# Autodesk Inventor assembly: T4DB 170
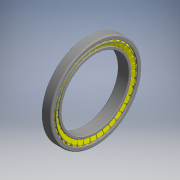
[picture p0: Inventor's stored thumbnail of the model, 180x180]
Saved by Autodesk Inventor 2017.3 (Build 213256000, 256)
## iProperties
Category: PARTsolutions
Company: SKF
Part Number: T4DB 170
Catalog Web Link: www.cadenas.de
Description: BT1_001_101-Tapered roller bearings, single row
Vendor: SKF
Document SubType Name: Assembly
Designer: partserver
Manufacturer: SKF
Mass: 3439 g
Surface Area: 1785.69 cm^2
Volume: 432.234 cm^3
Density: 7.95634 g/cm^3
Title: T4DB 170
Author: Cadenas PARTsolutions
Comments: Tapered roller bearings, single row
PSOL_IDENT_0: {$CADENAS_DATA\23d-libs\skf\bearings_units_and_housings\roller_bearings\tapered_roller_bearings\tape
PSOL_IDENT_1: red_roller_bearings_single_row\bt1_001_101.prj},177 {VTYP=3D},{STYP=ASSTAB},{NB=T4DB 170},{LINA=T4DB
PSOL_IDENT_2: 170},{NN=BT1_001_101},{DATE=23.12.2020 07:01:44},{GEOMDATE=30.11.2020 07:39:16},{VERSION=},{LINEID=
PSOL_IDENT_3: 4320},{WBVAR=},{WBNUMERIC=}  {NB=T4DB 170},{LINA=T4DB 170},{KT=DUMMY},{DESIGNATION=T4DB 170},{DD=170
PSOL_IDENT_4: .000},{D=230.000},{T=32.000},{DD1=197.5000},{D1=MIN},{ALPHA=17.100},{RANGLE=2.500},{IRA=14.600},{B=3
PSOL_IDENT_5: 0.000},{C=23.000},{C1=MIN},{R12=3.0},{R34=3.0},{AA=44.29541},{PITCH=200.033},{DW=16.450},{LW=21.500}
PSOL_IDENT_6: ,{DDAMAX=182},{DDAMIN=184.5},{DAMIN=215},{DAMAX=216.0},{DBMIN=223},{CA=6},{CB=9.0},{RA=3.0},{RB=3.0}
PSOL_IDENT_7: ,{LOAD1=307.000},{LOAD2=440.000},{LOAD3=43.000},{SPEED1=2000},{SPEED2=2600},{EE=0.46},{Y=1.30},{Y0=0
PSOL_IDENT_8: .7},{Y1=0},{X1=1},{X2=0.4},{X0=0.5},{Z=37},{II=1},{R1=0.00000231},{R2=10.9},{S1=0.019},{S2=2},{KZ=6}
PSOL_IDENT_9: ,{KL=0.7},{BF=2},{MASS=3.439},{DESIGN=trb1},{HELP=0.000},{PPATH=parts/bt1_001_101_asmtpl.prj},{SUPPR
PSOL_IDENT_10: ESS=N},{A4=200000},{A15=350000},{BEARING=T4DB 170},{A8=300000},{POPULAR=}
NB: T4DB 170
NN: BT1_001_101
NT: Tapered roller bearings, single row
NBSYN: $DESIGNATION.
LINA: T4DB 170
CATALOG: SKF
DESIGNATION: T4DB 170
DD: 170
D: 230
T: 32
LOAD1: 307
LOAD2: 440
LOAD3: 43
SPEED1: 2000
SPEED2: 2600
A4: 200000
A15: 350000
BEARING: T4DB 170
A8: 300000
SUPPLIER: SKF
ARTICLENO: T4DB 170
BOMINFO: T4DB 170
CREATOR: CADENAS GmbH
## Documents named in this file (5)
- e:\temp\worker_20\temp\exporttempdir_7356_2_3SxGk\format_0\T4DB 170.iam
- e:\temp\worker_20\temp\exporttempdir_7356_2_3SxGk\format_0\T4DB 170_ir.ipt
- e:\temp\worker_20\temp\exporttempdir_7356_2_3SxGk\format_0\T4DB 170_cage.ipt
- e:\temp\worker_20\temp\exporttempdir_7356_2_3SxGk\format_0\T4DB 170_r.ipt
- e:\temp\worker_20\temp\exporttempdir_7356_2_3SxGk\format_0\T4DB 170_or.ipt
## Components (40 placed, 4 different names)
1. T4DB 170_ir:1
2. T4DB 170_cage:1 — roller1_XY@2 <-> roller_XY@3, roller1_Z@2 <-> roller_Z@3, roller1_YZ@2 <-> roller_YZ@3, roller2_XY@2 <-> roller_XY@4, roller2_Z@2 <-> roller_Z@4, roller2_YZ@2 <-> roller_YZ@4, roller3_XY@2 <-> roller_XY@5, roller3_Z@2 <-> roller_Z@5, roller3_YZ@2 <-> roller_YZ@5, roller4_XY@2 <-> roller_XY@6, roller4_Z@2 <-> roller_Z@6, roller4_YZ@2 <-> roller_YZ@6, roller5_XY@2 <-> roller_XY@7, roller5_Z@2 <-> roller_Z@7, roller5_YZ@2 <-> roller_YZ@7, roller6_XY@2 <-> roller_XY@8, roller6_Z@2 <-> roller_Z@8, roller6_YZ@2 <-> roller_YZ@8, roller7_XY@2 <-> roller_XY@9, roller7_Z@2 <-> roller_Z@9, roller7_YZ@2 <-> roller_YZ@9, roller8_XY@2 <-> roller_XY@10, roller8_Z@2 <-> roller_Z@10, roller8_YZ@2 <-> roller_YZ@10, roller9_XY@2 <-> roller_XY@11, roller9_Z@2 <-> roller_Z@11, roller9_YZ@2 <-> roller_YZ@11, roller10_XY@2 <-> roller_XY@12, roller10_Z@2 <-> roller_Z@12, roller10_YZ@2 <-> roller_YZ@12, roller11_XY@2 <-> roller_XY@13, roller11_Z@2 <-> roller_Z@13, roller11_YZ@2 <-> roller_YZ@13, roller12_XY@2 <-> roller_XY@14, roller12_Z@2 <-> roller_Z@14, roller12_YZ@2 <-> roller_YZ@14, roller13_XY@2 <-> roller_XY@15, roller13_Z@2 <-> roller_Z@15, roller13_YZ@2 <-> roller_YZ@15, roller14_XY@2 <-> roller_XY@16, roller14_Z@2 <-> roller_Z@16, roller14_YZ@2 <-> roller_YZ@16, roller15_XY@2 <-> roller_XY@17, roller15_Z@2 <-> roller_Z@17, roller15_YZ@2 <-> roller_YZ@17, roller16_XY@2 <-> roller_XY@18, roller16_Z@2 <-> roller_Z@18, roller16_YZ@2 <-> roller_YZ@18, roller17_XY@2 <-> roller_XY@19, roller17_Z@2 <-> roller_Z@19, roller17_YZ@2 <-> roller_YZ@19, roller18_XY@2 <-> roller_XY@20, roller18_Z@2 <-> roller_Z@20, roller18_YZ@2 <-> roller_YZ@20, roller19_XY@2 <-> roller_XY@21, roller19_Z@2 <-> roller_Z@21, roller19_YZ@2 <-> roller_YZ@21, roller20_XY@2 <-> roller_XY@22, roller20_Z@2 <-> roller_Z@22, roller20_YZ@2 <-> roller_YZ@22, roller21_XY@2 <-> roller_XY@23, roller21_Z@2 <-> roller_Z@23, roller21_YZ@2 <-> roller_YZ@23, roller22_XY@2 <-> roller_XY@24, roller22_Z@2 <-> roller_Z@24, roller22_YZ@2 <-> roller_YZ@24, roller23_XY@2 <-> roller_XY@25, roller23_Z@2 <-> roller_Z@25, roller23_YZ@2 <-> roller_YZ@25, roller24_XY@2 <-> roller_XY@26, roller24_Z@2 <-> roller_Z@26, roller24_YZ@2 <-> roller_YZ@26, roller25_XY@2 <-> roller_XY@27, roller25_Z@2 <-> roller_Z@27, roller25_YZ@2 <-> roller_YZ@27, roller26_XY@2 <-> roller_XY@28, roller26_Z@2 <-> roller_Z@28, roller26_YZ@2 <-> roller_YZ@28, roller27_XY@2 <-> roller_XY@29, roller27_Z@2 <-> roller_Z@29, roller27_YZ@2 <-> roller_YZ@29, roller28_XY@2 <-> roller_XY@30, roller28_Z@2 <-> roller_Z@30, roller28_YZ@2 <-> roller_YZ@30, roller29_XY@2 <-> roller_XY@31, roller29_Z@2 <-> roller_Z@31, roller29_YZ@2 <-> roller_YZ@31, roller30_XY@2 <-> roller_XY@32, roller30_Z@2 <-> roller_Z@32, roller30_YZ@2 <-> roller_YZ@32, roller31_XY@2 <-> roller_XY@33, roller31_Z@2 <-> roller_Z@33, roller31_YZ@2 <-> roller_YZ@33, roller32_XY@2 <-> roller_XY@34, roller32_Z@2 <-> roller_Z@34, roller32_YZ@2 <-> roller_YZ@34, roller33_XY@2 <-> roller_XY@35, roller33_Z@2 <-> roller_Z@35, roller33_YZ@2 <-> roller_YZ@35, roller34_XY@2 <-> roller_XY@36, roller34_Z@2 <-> roller_Z@36, roller34_YZ@2 <-> roller_YZ@36, roller35_XY@2 <-> roller_XY@37, roller35_Z@2 <-> roller_Z@37, roller35_YZ@2 <-> roller_YZ@37, roller36_XY@2 <-> roller_XY@38, roller36_Z@2 <-> roller_Z@38, roller36_YZ@2 <-> roller_YZ@38, roller37_XY@2 <-> roller_XY@39, roller37_Z@2 <-> roller_Z@39, roller37_YZ@2 <-> roller_YZ@39
3. T4DB 170_r:1 — roller1_XY@2 <-> roller_XY@3, roller1_Z@2 <-> roller_Z@3, roller1_YZ@2 <-> roller_YZ@3
4. T4DB 170_r:2 — roller2_XY@2 <-> roller_XY@4, roller2_Z@2 <-> roller_Z@4, roller2_YZ@2 <-> roller_YZ@4
5. T4DB 170_r:3 — roller3_XY@2 <-> roller_XY@5, roller3_Z@2 <-> roller_Z@5, roller3_YZ@2 <-> roller_YZ@5
6. T4DB 170_r:4 — roller4_XY@2 <-> roller_XY@6, roller4_Z@2 <-> roller_Z@6, roller4_YZ@2 <-> roller_YZ@6
7. T4DB 170_r:5 — roller5_XY@2 <-> roller_XY@7, roller5_Z@2 <-> roller_Z@7, roller5_YZ@2 <-> roller_YZ@7
8. T4DB 170_r:6 — roller6_XY@2 <-> roller_XY@8, roller6_Z@2 <-> roller_Z@8, roller6_YZ@2 <-> roller_YZ@8
9. T4DB 170_r:7 — roller7_XY@2 <-> roller_XY@9, roller7_Z@2 <-> roller_Z@9, roller7_YZ@2 <-> roller_YZ@9
10. T4DB 170_r:8 — roller8_XY@2 <-> roller_XY@10, roller8_Z@2 <-> roller_Z@10, roller8_YZ@2 <-> roller_YZ@10
11. T4DB 170_r:9 — roller9_XY@2 <-> roller_XY@11, roller9_Z@2 <-> roller_Z@11, roller9_YZ@2 <-> roller_YZ@11
12. T4DB 170_r:10 — roller10_XY@2 <-> roller_XY@12, roller10_Z@2 <-> roller_Z@12, roller10_YZ@2 <-> roller_YZ@12
13. T4DB 170_r:11 — roller11_XY@2 <-> roller_XY@13, roller11_Z@2 <-> roller_Z@13, roller11_YZ@2 <-> roller_YZ@13
14. T4DB 170_r:12 — roller12_XY@2 <-> roller_XY@14, roller12_Z@2 <-> roller_Z@14, roller12_YZ@2 <-> roller_YZ@14
15. T4DB 170_r:13 — roller13_XY@2 <-> roller_XY@15, roller13_Z@2 <-> roller_Z@15, roller13_YZ@2 <-> roller_YZ@15
16. T4DB 170_r:14 — roller14_XY@2 <-> roller_XY@16, roller14_Z@2 <-> roller_Z@16, roller14_YZ@2 <-> roller_YZ@16
17. T4DB 170_r:15 — roller15_XY@2 <-> roller_XY@17, roller15_Z@2 <-> roller_Z@17, roller15_YZ@2 <-> roller_YZ@17
18. T4DB 170_r:16 — roller16_XY@2 <-> roller_XY@18, roller16_Z@2 <-> roller_Z@18, roller16_YZ@2 <-> roller_YZ@18
19. T4DB 170_r:17 — roller17_XY@2 <-> roller_XY@19, roller17_Z@2 <-> roller_Z@19, roller17_YZ@2 <-> roller_YZ@19
20. T4DB 170_r:18 — roller18_XY@2 <-> roller_XY@20, roller18_Z@2 <-> roller_Z@20, roller18_YZ@2 <-> roller_YZ@20
21. T4DB 170_r:19 — roller19_XY@2 <-> roller_XY@21, roller19_Z@2 <-> roller_Z@21, roller19_YZ@2 <-> roller_YZ@21
22. T4DB 170_r:20 — roller20_XY@2 <-> roller_XY@22, roller20_Z@2 <-> roller_Z@22, roller20_YZ@2 <-> roller_YZ@22
23. T4DB 170_r:21 — roller21_XY@2 <-> roller_XY@23, roller21_Z@2 <-> roller_Z@23, roller21_YZ@2 <-> roller_YZ@23
24. T4DB 170_r:22 — roller22_XY@2 <-> roller_XY@24, roller22_Z@2 <-> roller_Z@24, roller22_YZ@2 <-> roller_YZ@24
25. T4DB 170_r:23 — roller23_XY@2 <-> roller_XY@25, roller23_Z@2 <-> roller_Z@25, roller23_YZ@2 <-> roller_YZ@25
26. T4DB 170_r:24 — roller24_XY@2 <-> roller_XY@26, roller24_Z@2 <-> roller_Z@26, roller24_YZ@2 <-> roller_YZ@26
27. T4DB 170_r:25 — roller25_XY@2 <-> roller_XY@27, roller25_Z@2 <-> roller_Z@27, roller25_YZ@2 <-> roller_YZ@27
28. T4DB 170_r:26 — roller26_XY@2 <-> roller_XY@28, roller26_Z@2 <-> roller_Z@28, roller26_YZ@2 <-> roller_YZ@28
29. T4DB 170_r:27 — roller27_XY@2 <-> roller_XY@29, roller27_Z@2 <-> roller_Z@29, roller27_YZ@2 <-> roller_YZ@29
30. T4DB 170_r:28 — roller28_XY@2 <-> roller_XY@30, roller28_Z@2 <-> roller_Z@30, roller28_YZ@2 <-> roller_YZ@30
31. T4DB 170_r:29 — roller29_XY@2 <-> roller_XY@31, roller29_Z@2 <-> roller_Z@31, roller29_YZ@2 <-> roller_YZ@31
32. T4DB 170_r:30 — roller30_XY@2 <-> roller_XY@32, roller30_Z@2 <-> roller_Z@32, roller30_YZ@2 <-> roller_YZ@32
33. T4DB 170_r:31 — roller31_XY@2 <-> roller_XY@33, roller31_Z@2 <-> roller_Z@33, roller31_YZ@2 <-> roller_YZ@33
34. T4DB 170_r:32 — roller32_XY@2 <-> roller_XY@34, roller32_Z@2 <-> roller_Z@34, roller32_YZ@2 <-> roller_YZ@34
35. T4DB 170_r:33 — roller33_XY@2 <-> roller_XY@35, roller33_Z@2 <-> roller_Z@35, roller33_YZ@2 <-> roller_YZ@35
36. T4DB 170_r:34 — roller34_XY@2 <-> roller_XY@36, roller34_Z@2 <-> roller_Z@36, roller34_YZ@2 <-> roller_YZ@36
37. T4DB 170_r:35 — roller35_XY@2 <-> roller_XY@37, roller35_Z@2 <-> roller_Z@37, roller35_YZ@2 <-> roller_YZ@37
38. T4DB 170_r:36 — roller36_XY@2 <-> roller_XY@38, roller36_Z@2 <-> roller_Z@38, roller36_YZ@2 <-> roller_YZ@38
39. T4DB 170_r:37 — roller37_XY@2 <-> roller_XY@39, roller37_Z@2 <-> roller_Z@39, roller37_YZ@2 <-> roller_YZ@39
40. T4DB 170_or:1
## Relationships (111: Mate 74, Angle 37)
- roller1_XY@2 <-> roller_XY@3 [Mate]: T4DB 170_cage:1 ↔ T4DB 170_r:1
- roller1_Z@2 <-> roller_Z@3 [Mate]: T4DB 170_cage:1 ↔ T4DB 170_r:1
- roller1_YZ@2 <-> roller_YZ@3 [Angle] (0 deg): T4DB 170_cage:1 ↔ T4DB 170_r:1
- roller2_XY@2 <-> roller_XY@4 [Mate]: T4DB 170_cage:1 ↔ T4DB 170_r:2
- roller2_Z@2 <-> roller_Z@4 [Mate]: T4DB 170_cage:1 ↔ T4DB 170_r:2
- roller2_YZ@2 <-> roller_YZ@4 [Angle] (0 deg): T4DB 170_cage:1 ↔ T4DB 170_r:2
- roller3_XY@2 <-> roller_XY@5 [Mate]: T4DB 170_cage:1 ↔ T4DB 170_r:3
- roller3_Z@2 <-> roller_Z@5 [Mate]: T4DB 170_cage:1 ↔ T4DB 170_r:3
- roller3_YZ@2 <-> roller_YZ@5 [Angle] (0 deg): T4DB 170_cage:1 ↔ T4DB 170_r:3
- roller4_XY@2 <-> roller_XY@6 [Mate]: T4DB 170_cage:1 ↔ T4DB 170_r:4
- roller4_Z@2 <-> roller_Z@6 [Mate]: T4DB 170_cage:1 ↔ T4DB 170_r:4
- roller4_YZ@2 <-> roller_YZ@6 [Angle] (0 deg): T4DB 170_cage:1 ↔ T4DB 170_r:4
- roller5_XY@2 <-> roller_XY@7 [Mate]: T4DB 170_cage:1 ↔ T4DB 170_r:5
- roller5_Z@2 <-> roller_Z@7 [Mate]: T4DB 170_cage:1 ↔ T4DB 170_r:5
- roller5_YZ@2 <-> roller_YZ@7 [Angle] (0 deg): T4DB 170_cage:1 ↔ T4DB 170_r:5
- roller6_XY@2 <-> roller_XY@8 [Mate]: T4DB 170_cage:1 ↔ T4DB 170_r:6
- roller6_Z@2 <-> roller_Z@8 [Mate]: T4DB 170_cage:1 ↔ T4DB 170_r:6
- roller6_YZ@2 <-> roller_YZ@8 [Angle] (0 deg): T4DB 170_cage:1 ↔ T4DB 170_r:6
- roller7_XY@2 <-> roller_XY@9 [Mate]: T4DB 170_cage:1 ↔ T4DB 170_r:7
- roller7_Z@2 <-> roller_Z@9 [Mate]: T4DB 170_cage:1 ↔ T4DB 170_r:7
- roller7_YZ@2 <-> roller_YZ@9 [Angle] (0 deg): T4DB 170_cage:1 ↔ T4DB 170_r:7
- roller8_XY@2 <-> roller_XY@10 [Mate]: T4DB 170_cage:1 ↔ T4DB 170_r:8
- roller8_Z@2 <-> roller_Z@10 [Mate]: T4DB 170_cage:1 ↔ T4DB 170_r:8
- roller8_YZ@2 <-> roller_YZ@10 [Angle] (0 deg): T4DB 170_cage:1 ↔ T4DB 170_r:8
- roller9_XY@2 <-> roller_XY@11 [Mate]: T4DB 170_cage:1 ↔ T4DB 170_r:9
- roller9_Z@2 <-> roller_Z@11 [Mate]: T4DB 170_cage:1 ↔ T4DB 170_r:9
- roller9_YZ@2 <-> roller_YZ@11 [Angle] (0 deg): T4DB 170_cage:1 ↔ T4DB 170_r:9
- roller10_XY@2 <-> roller_XY@12 [Mate]: T4DB 170_cage:1 ↔ T4DB 170_r:10
- roller10_Z@2 <-> roller_Z@12 [Mate]: T4DB 170_cage:1 ↔ T4DB 170_r:10
- roller10_YZ@2 <-> roller_YZ@12 [Angle] (0 deg): T4DB 170_cage:1 ↔ T4DB 170_r:10
- roller11_XY@2 <-> roller_XY@13 [Mate]: T4DB 170_cage:1 ↔ T4DB 170_r:11
- roller11_Z@2 <-> roller_Z@13 [Mate]: T4DB 170_cage:1 ↔ T4DB 170_r:11
- roller11_YZ@2 <-> roller_YZ@13 [Angle] (0 deg): T4DB 170_cage:1 ↔ T4DB 170_r:11
- roller12_XY@2 <-> roller_XY@14 [Mate]: T4DB 170_cage:1 ↔ T4DB 170_r:12
- roller12_Z@2 <-> roller_Z@14 [Mate]: T4DB 170_cage:1 ↔ T4DB 170_r:12
- roller12_YZ@2 <-> roller_YZ@14 [Angle] (0 deg): T4DB 170_cage:1 ↔ T4DB 170_r:12
- roller13_XY@2 <-> roller_XY@15 [Mate]: T4DB 170_cage:1 ↔ T4DB 170_r:13
- roller13_Z@2 <-> roller_Z@15 [Mate]: T4DB 170_cage:1 ↔ T4DB 170_r:13
- roller13_YZ@2 <-> roller_YZ@15 [Angle] (0 deg): T4DB 170_cage:1 ↔ T4DB 170_r:13
- roller14_XY@2 <-> roller_XY@16 [Mate]: T4DB 170_cage:1 ↔ T4DB 170_r:14
- roller14_Z@2 <-> roller_Z@16 [Mate]: T4DB 170_cage:1 ↔ T4DB 170_r:14
- roller14_YZ@2 <-> roller_YZ@16 [Angle] (0 deg): T4DB 170_cage:1 ↔ T4DB 170_r:14
- roller15_XY@2 <-> roller_XY@17 [Mate]: T4DB 170_cage:1 ↔ T4DB 170_r:15
- roller15_Z@2 <-> roller_Z@17 [Mate]: T4DB 170_cage:1 ↔ T4DB 170_r:15
- roller15_YZ@2 <-> roller_YZ@17 [Angle] (0 deg): T4DB 170_cage:1 ↔ T4DB 170_r:15
- roller16_XY@2 <-> roller_XY@18 [Mate]: T4DB 170_cage:1 ↔ T4DB 170_r:16
- roller16_Z@2 <-> roller_Z@18 [Mate]: T4DB 170_cage:1 ↔ T4DB 170_r:16
- roller16_YZ@2 <-> roller_YZ@18 [Angle] (0 deg): T4DB 170_cage:1 ↔ T4DB 170_r:16
- roller17_XY@2 <-> roller_XY@19 [Mate]: T4DB 170_cage:1 ↔ T4DB 170_r:17
- roller17_Z@2 <-> roller_Z@19 [Mate]: T4DB 170_cage:1 ↔ T4DB 170_r:17
- roller17_YZ@2 <-> roller_YZ@19 [Angle] (0 deg): T4DB 170_cage:1 ↔ T4DB 170_r:17
- roller18_XY@2 <-> roller_XY@20 [Mate]: T4DB 170_cage:1 ↔ T4DB 170_r:18
- roller18_Z@2 <-> roller_Z@20 [Mate]: T4DB 170_cage:1 ↔ T4DB 170_r:18
- roller18_YZ@2 <-> roller_YZ@20 [Angle] (0 deg): T4DB 170_cage:1 ↔ T4DB 170_r:18
- roller19_XY@2 <-> roller_XY@21 [Mate]: T4DB 170_cage:1 ↔ T4DB 170_r:19
- roller19_Z@2 <-> roller_Z@21 [Mate]: T4DB 170_cage:1 ↔ T4DB 170_r:19
- roller19_YZ@2 <-> roller_YZ@21 [Angle] (0 deg): T4DB 170_cage:1 ↔ T4DB 170_r:19
- roller20_XY@2 <-> roller_XY@22 [Mate]: T4DB 170_cage:1 ↔ T4DB 170_r:20
- roller20_Z@2 <-> roller_Z@22 [Mate]: T4DB 170_cage:1 ↔ T4DB 170_r:20
- roller20_YZ@2 <-> roller_YZ@22 [Angle] (0 deg): T4DB 170_cage:1 ↔ T4DB 170_r:20
- roller21_XY@2 <-> roller_XY@23 [Mate]: T4DB 170_cage:1 ↔ T4DB 170_r:21
- roller21_Z@2 <-> roller_Z@23 [Mate]: T4DB 170_cage:1 ↔ T4DB 170_r:21
- roller21_YZ@2 <-> roller_YZ@23 [Angle] (0 deg): T4DB 170_cage:1 ↔ T4DB 170_r:21
- roller22_XY@2 <-> roller_XY@24 [Mate]: T4DB 170_cage:1 ↔ T4DB 170_r:22
- roller22_Z@2 <-> roller_Z@24 [Mate]: T4DB 170_cage:1 ↔ T4DB 170_r:22
- roller22_YZ@2 <-> roller_YZ@24 [Angle] (0 deg): T4DB 170_cage:1 ↔ T4DB 170_r:22
- roller23_XY@2 <-> roller_XY@25 [Mate]: T4DB 170_cage:1 ↔ T4DB 170_r:23
- roller23_Z@2 <-> roller_Z@25 [Mate]: T4DB 170_cage:1 ↔ T4DB 170_r:23
- roller23_YZ@2 <-> roller_YZ@25 [Angle] (0 deg): T4DB 170_cage:1 ↔ T4DB 170_r:23
- roller24_XY@2 <-> roller_XY@26 [Mate]: T4DB 170_cage:1 ↔ T4DB 170_r:24
- roller24_Z@2 <-> roller_Z@26 [Mate]: T4DB 170_cage:1 ↔ T4DB 170_r:24
- roller24_YZ@2 <-> roller_YZ@26 [Angle] (0 deg): T4DB 170_cage:1 ↔ T4DB 170_r:24
- roller25_XY@2 <-> roller_XY@27 [Mate]: T4DB 170_cage:1 ↔ T4DB 170_r:25
- roller25_Z@2 <-> roller_Z@27 [Mate]: T4DB 170_cage:1 ↔ T4DB 170_r:25
- roller25_YZ@2 <-> roller_YZ@27 [Angle] (0 deg): T4DB 170_cage:1 ↔ T4DB 170_r:25
- roller26_XY@2 <-> roller_XY@28 [Mate]: T4DB 170_cage:1 ↔ T4DB 170_r:26
- roller26_Z@2 <-> roller_Z@28 [Mate]: T4DB 170_cage:1 ↔ T4DB 170_r:26
- roller26_YZ@2 <-> roller_YZ@28 [Angle] (0 deg): T4DB 170_cage:1 ↔ T4DB 170_r:26
- roller27_XY@2 <-> roller_XY@29 [Mate]: T4DB 170_cage:1 ↔ T4DB 170_r:27
- roller27_Z@2 <-> roller_Z@29 [Mate]: T4DB 170_cage:1 ↔ T4DB 170_r:27
- roller27_YZ@2 <-> roller_YZ@29 [Angle] (0 deg): T4DB 170_cage:1 ↔ T4DB 170_r:27
- roller28_XY@2 <-> roller_XY@30 [Mate]: T4DB 170_cage:1 ↔ T4DB 170_r:28
- roller28_Z@2 <-> roller_Z@30 [Mate]: T4DB 170_cage:1 ↔ T4DB 170_r:28
- roller28_YZ@2 <-> roller_YZ@30 [Angle] (0 deg): T4DB 170_cage:1 ↔ T4DB 170_r:28
- roller29_XY@2 <-> roller_XY@31 [Mate]: T4DB 170_cage:1 ↔ T4DB 170_r:29
- roller29_Z@2 <-> roller_Z@31 [Mate]: T4DB 170_cage:1 ↔ T4DB 170_r:29
- roller29_YZ@2 <-> roller_YZ@31 [Angle] (0 deg): T4DB 170_cage:1 ↔ T4DB 170_r:29
- roller30_XY@2 <-> roller_XY@32 [Mate]: T4DB 170_cage:1 ↔ T4DB 170_r:30
- roller30_Z@2 <-> roller_Z@32 [Mate]: T4DB 170_cage:1 ↔ T4DB 170_r:30
- roller30_YZ@2 <-> roller_YZ@32 [Angle] (0 deg): T4DB 170_cage:1 ↔ T4DB 170_r:30
- roller31_XY@2 <-> roller_XY@33 [Mate]: T4DB 170_cage:1 ↔ T4DB 170_r:31
- roller31_Z@2 <-> roller_Z@33 [Mate]: T4DB 170_cage:1 ↔ T4DB 170_r:31
- roller31_YZ@2 <-> roller_YZ@33 [Angle] (0 deg): T4DB 170_cage:1 ↔ T4DB 170_r:31
- roller32_XY@2 <-> roller_XY@34 [Mate]: T4DB 170_cage:1 ↔ T4DB 170_r:32
- roller32_Z@2 <-> roller_Z@34 [Mate]: T4DB 170_cage:1 ↔ T4DB 170_r:32
- roller32_YZ@2 <-> roller_YZ@34 [Angle] (0 deg): T4DB 170_cage:1 ↔ T4DB 170_r:32
- roller33_XY@2 <-> roller_XY@35 [Mate]: T4DB 170_cage:1 ↔ T4DB 170_r:33
- roller33_Z@2 <-> roller_Z@35 [Mate]: T4DB 170_cage:1 ↔ T4DB 170_r:33
- roller33_YZ@2 <-> roller_YZ@35 [Angle] (0 deg): T4DB 170_cage:1 ↔ T4DB 170_r:33
- roller34_XY@2 <-> roller_XY@36 [Mate]: T4DB 170_cage:1 ↔ T4DB 170_r:34
- roller34_Z@2 <-> roller_Z@36 [Mate]: T4DB 170_cage:1 ↔ T4DB 170_r:34
- roller34_YZ@2 <-> roller_YZ@36 [Angle] (0 deg): T4DB 170_cage:1 ↔ T4DB 170_r:34
- roller35_XY@2 <-> roller_XY@37 [Mate]: T4DB 170_cage:1 ↔ T4DB 170_r:35
- roller35_Z@2 <-> roller_Z@37 [Mate]: T4DB 170_cage:1 ↔ T4DB 170_r:35
- roller35_YZ@2 <-> roller_YZ@37 [Angle] (0 deg): T4DB 170_cage:1 ↔ T4DB 170_r:35
- roller36_XY@2 <-> roller_XY@38 [Mate]: T4DB 170_cage:1 ↔ T4DB 170_r:36
- roller36_Z@2 <-> roller_Z@38 [Mate]: T4DB 170_cage:1 ↔ T4DB 170_r:36
- roller36_YZ@2 <-> roller_YZ@38 [Angle] (0 deg): T4DB 170_cage:1 ↔ T4DB 170_r:36
- roller37_XY@2 <-> roller_XY@39 [Mate]: T4DB 170_cage:1 ↔ T4DB 170_r:37
- roller37_Z@2 <-> roller_Z@39 [Mate]: T4DB 170_cage:1 ↔ T4DB 170_r:37
- roller37_YZ@2 <-> roller_YZ@39 [Angle] (0 deg): T4DB 170_cage:1 ↔ T4DB 170_r:37
